# Autodesk Inventor assembly: ir+marco
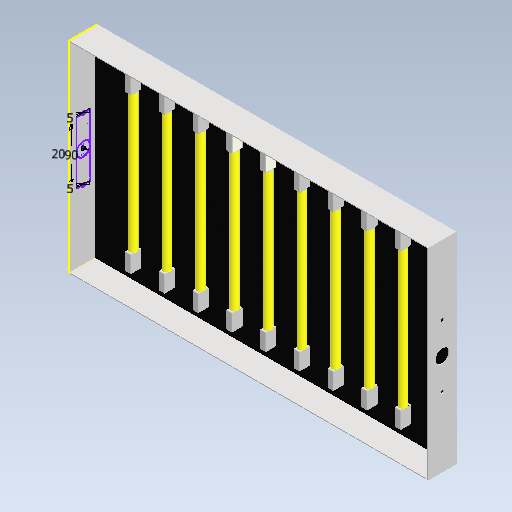
[picture p0: Inventor's stored thumbnail of the model, 512x512]
Saved by Autodesk Inventor 2021 (Build 250183000, 183)
## iProperties
Created: 2021-11-08
Part Number: ir+marco
Document SubType Name: Assembly
Designer: arthu
Author: arthu
## Documents named in this file (4)
- C:\Users\arthu\OneDrive\Escritorio\TersusMax\ir_cafe\ir+marco.iam
- C:\Users\arthu\OneDrive\Escritorio\TersusMax\ir_cafe\marco_ir.ipt
- C:\Users\arthu\OneDrive\Escritorio\TersusMax\ir_cafe\vidrio_ir.ipt
- C:\Users\arthu\OneDrive\Escritorio\TersusMax\ir_cafe\IR.ipt
## Components (11 placed, 3 different names)
1. marco_ir:1 — Rígido:1
2. vidrio_ir:1 — Rígido:1, Corredera:1
3. IR:1 — Corredera:1, Rígido:2, Rígido:6
4. IR:2 — Rígido:2, Rígido:3
5. IR:3 — Rígido:6, Rígido:7
6. IR:4 — Rígido:5
7. IR:5 — Rígido:4, Rígido:5
8. IR:6 — Rígido:3, Rígido:4
9. IR:7 — Rígido:7, Rígido:8
10. IR:8 — Rígido:8, Rígido:9
11. IR:9 — Rígido:9
## Relationships (10: WeldJoint 9, TranslationJoint 1)
- Rígido:1 [WeldJoint]: marco_ir:1 ↔ vidrio_ir:1
- Corredera:1 [TranslationJoint]: vidrio_ir:1 ↔ IR:1
- Rígido:2 [WeldJoint] (40 mm): IR:1 ↔ IR:2
- Rígido:3 [WeldJoint] (40 mm): IR:2 ↔ IR:6
- Rígido:4 [WeldJoint] (40 mm): IR:5 ↔ IR:6
- Rígido:5 [WeldJoint] (40 mm): IR:4 ↔ IR:5
- Rígido:6 [WeldJoint] (40 mm): IR:1 ↔ IR:3
- Rígido:7 [WeldJoint] (40 mm): IR:3 ↔ IR:7
- Rígido:8 [WeldJoint] (40 mm): IR:7 ↔ IR:8
- Rígido:9 [WeldJoint] (40 mm): IR:8 ↔ IR:9
